# Autodesk Inventor assembly: shamisen
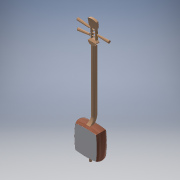
[picture p0: Inventor's stored thumbnail of the model, 180x180]
Saved by Autodesk Inventor 2019 (Build 230136000, 136)
## iProperties
Created: 2019-11-15
Part Number: shamisen
Material: Типовые
Document SubType Name: Assembly
Designer: stepa
Mass: 1027.05 g
Surface Area: 4415.24 cm^2
Volume: 1631.57 cm^3
Density: 0.629485 g/cm^3
Author: stepa
## Documents named in this file (11)
- C:\Users\stepa\Documents\Inventor\Shamisen\shamisen.iam
- C:\Users\stepa\Documents\Inventor\Shamisen\dou_long.ipt
- C:\Users\stepa\Documents\Inventor\Shamisen\dou_short_round.ipt
- C:\Users\stepa\Documents\Inventor\Shamisen\dou_short_square.ipt
- C:\Users\stepa\Documents\Inventor\Shamisen\sao.ipt
- C:\Users\stepa\Documents\Inventor\Shamisen\nakagi.ipt
- C:\Users\stepa\Documents\Inventor\Shamisen\tenjin.ipt
- C:\Users\stepa\Documents\Inventor\Shamisen\hole_big.ipt
- C:\Users\stepa\Documents\Inventor\Shamisen\hole_small.ipt
- C:\Users\stepa\Documents\Inventor\Shamisen\itomaki.ipt
- C:\Users\stepa\Documents\Inventor\Shamisen\kawa.ipt
## Components (18 placed, 10 different names)
1. dou_long:1 — Заподлицо:1, Совмещение:1, Заподлицо:4, Совмещение:4
2. dou_long:2 — Заподлицо:2, Заподлицо:3, Совмещение:2, Совмещение:3
3. dou_short_round:1 — Заподлицо:1, Совмещение:1, Заподлицо:2, Совмещение:2, Совмещение:9, Совмещение:23
4. dou_short_square:1 — Заподлицо:3, Заподлицо:4, Совмещение:3, Совмещение:4, Совмещение:7, Совмещение:8, Совмещение:22
5. sao:1 — Совмещение:5, Совмещение:6, Заподлицо:5, Совмещение:7, Совмещение:8, Заподлицо:6, Заподлицо:7, Совмещение:10
6. nakagi:1 — Совмещение:5, Совмещение:6, Заподлицо:5, Совмещение:9
7. tenjin:1 — Заподлицо:6, Заподлицо:7, Совмещение:10, Совмещение:11, Совмещение:12, Совмещение:13, Совмещение:14, Совмещение:15, Совмещение:16, Совмещение:17, Совмещение:18
8. hole_big:1 — Совмещение:11
9. hole_big:2 — Совмещение:12
10. hole_big:3 — Совмещение:13, Совмещение:14
11. hole_small:1 — Совмещение:16, Совмещение:19
12. hole_small:2 — Совмещение:17, Совмещение:20
13. hole_small:3 — Совмещение:15, Совмещение:18, Совмещение:21
14. itomaki:1 — Совмещение:21
15. itomaki:2 — Совмещение:19
16. itomaki:3 — Совмещение:20
17. kawa:1 — Совмещение:22
18. kawa:2 — Совмещение:23
## Relationships (30: Mate 23, Flush 7)
- Заподлицо:1 [Flush]: dou_long:1 ↔ dou_short_round:1
- Совмещение:1 [Mate]: dou_long:1 ↔ dou_short_round:1
- Заподлицо:2 [Flush]: dou_long:2 ↔ dou_short_round:1
- Заподлицо:3 [Flush]: dou_long:2 ↔ dou_short_square:1
- Заподлицо:4 [Flush]: dou_long:1 ↔ dou_short_square:1
- Совмещение:2 [Mate]: dou_long:2 ↔ dou_short_round:1
- Совмещение:3 [Mate]: dou_long:2 ↔ dou_short_square:1
- Совмещение:4 [Mate]: dou_long:1 ↔ dou_short_square:1
- Совмещение:5 [Mate]: sao:1 ↔ nakagi:1
- Совмещение:6 [Mate]: sao:1 ↔ nakagi:1
- Заподлицо:5 [Flush]: sao:1 ↔ nakagi:1
- Совмещение:7 [Mate]: dou_short_square:1 ↔ sao:1
- Совмещение:8 [Mate]: dou_short_square:1 ↔ sao:1
- Совмещение:9 [Mate]: dou_short_round:1 ↔ nakagi:1
- Заподлицо:6 [Flush]: sao:1 ↔ tenjin:1
- Заподлицо:7 [Flush]: sao:1 ↔ tenjin:1
- Совмещение:10 [Mate]: sao:1 ↔ tenjin:1
- Совмещение:11 [Mate]: tenjin:1 ↔ hole_big:1
- Совмещение:12 [Mate]: tenjin:1 ↔ hole_big:2
- Совмещение:13 [Mate]: tenjin:1 ↔ hole_big:3
- Совмещение:14 [Mate]: tenjin:1 ↔ hole_big:3
- Совмещение:15 [Mate]: tenjin:1 ↔ hole_small:3
- Совмещение:16 [Mate]: tenjin:1 ↔ hole_small:1
- Совмещение:17 [Mate]: tenjin:1 ↔ hole_small:2
- Совмещение:18 [Mate]: tenjin:1 ↔ hole_small:3
- Совмещение:19 [Mate]: hole_small:1 ↔ itomaki:2
- Совмещение:20 [Mate]: hole_small:2 ↔ itomaki:3
- Совмещение:21 [Mate]: hole_small:3 ↔ itomaki:1
- Совмещение:22 [Mate]: dou_short_square:1 ↔ kawa:1
- Совмещение:23 [Mate]: dou_short_round:1 ↔ kawa:2
